# Autodesk Inventor assembly: adapt
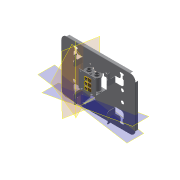
[picture p0: Inventor's stored thumbnail of the model, 180x180]
Saved by Autodesk Inventor 2022 (Build 260148000, 148)
## iProperties
Shininess: 64.0
Length Units: 11272
Angle Units: 11279
Time Units: 11290
Mass Units: 11286
Length Display Precision: 3
Angle Display Precision: 2
Created: 2002-05-01
Part Number: adapt
Document SubType Name: Assembly
Designer: Administrator
Density: 0.0
Volumn: 0.0
Area: 0.0
PropertySet Name: Model Information
Control State: 0
Master: False
Checked Out: False
Author: Administrator
## Documents named in this file (6)
- C:\Autodesk Inventor 2022 Advanced Assembly Modeling Practice Files\adapt.iam
- C:\Autodesk Inventor 2022 Advanced Assembly Modeling Practice Files\fishpaper.ipt
- C:\Autodesk Inventor 2022 Advanced Assembly Modeling Practice Files\contact.ipt
- C:\Autodesk Inventor 2022 Advanced Assembly Modeling Practice Files\6-32bolt.ipt
- C:\Autodesk Inventor 2022 Advanced Assembly Modeling Practice Files\coil.iam
- C:\Autodesk Inventor 2022 Advanced Assembly Modeling Practice Files\doorbellbase.ipt
## Components (10 placed, 5 different names)
1. doorbellbase:1 — Mate:2, Mate:3, Mate:4, Mate:5, Mate:6, Mate:7, Mate:13, Mate:14, Mate:15, Mate:16, Insert:7, Insert:8, Mate:21
2. fishpaper:1 — Mate:1, Mate:2, Mate:3, Insert:6, Mate:21
3. coil:1 [sub-assembly] — Insert:8
4. coil:2 [sub-assembly] — Insert:7
5. contact:1 — Mate:1, Insert:1, Insert:6
6. 6-32bolt:1 — Insert:1
7. contact:4
8. 6-32bolt:2
9. contact:5
10. 6-32bolt:3
## Component patterns: (3 elements, first: contact:1 + 6-32bolt:1)
## Relationships (20: Mate 16, Insert 4)
- Mate:1: fishpaper:1 ↔ contact:1
- Insert:1: contact:1 ↔ 6-32bolt:1
- Mate:2: doorbellbase:1 ↔ fishpaper:1
- Mate:3: doorbellbase:1 ↔ fishpaper:1
- Mate:4: doorbellbase:1
- Mate:5: doorbellbase:1
- Mate:6: doorbellbase:1
- Mate:7: doorbellbase:1
- Mate:8
- Mate:9
- Mate:13: doorbellbase:1
- Mate:14: doorbellbase:1
- Mate:15: doorbellbase:1
- Mate:16: doorbellbase:1
- Mate:17
- Mate:18
- Insert:6: fishpaper:1 ↔ contact:1
- Insert:7: doorbellbase:1 ↔ coil:2
- Insert:8: doorbellbase:1 ↔ coil:1
- Mate:21 (0.635 mm): doorbellbase:1 ↔ fishpaper:1
